# Autodesk Inventor assembly: rear_sled_MIR
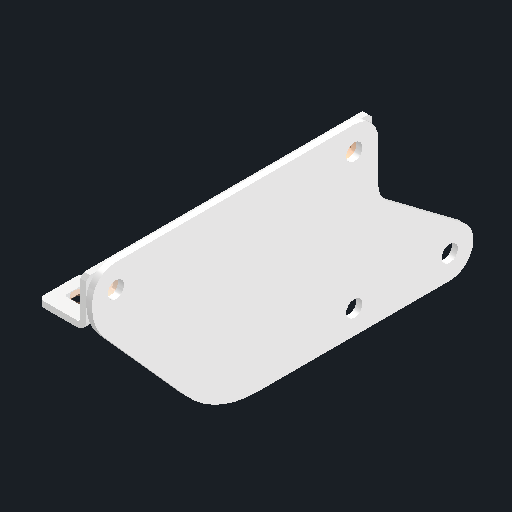
[picture p0: Inventor's stored thumbnail of the model, 512x512]
Saved by Autodesk Inventor 2024 (Build 280153000, 153)
## iProperties
Created: 2024-01-16
Part Number: rear_sled_MIR
Document SubType Name: Assembly
Designer: avere
Author: avere
## Documents named in this file (3)
- C:\Users\avere\Documents\rbp_cad\zoomba_v0.3\chassis\mirrored_parts\rear_sled_MIR.iam
- C:\Users\avere\Documents\rbp_cad\zoomba_v0.3\chassis\mirrored_parts\sled_MIR.ipt
- C:\Users\avere\Documents\rbp_cad\zoomba_v0.3\chassis\mirrored_parts\Alu Angle 1x1x6_MIR.ipt
## Components (2 placed, 2 different names)
1. sled_MIR:1 — Mate:1, Insert:1
2. Alu Angle 1x1x6_MIR:1 — Mate:1, Insert:1
## Relationships (2: Mate 1, Insert 1)
- Mate:1: sled_MIR:1 ↔ Alu Angle 1x1x6_MIR:1
- Insert:1: sled_MIR:1 ↔ Alu Angle 1x1x6_MIR:1
